# Autodesk Inventor assembly: HighFlowCO2Laser
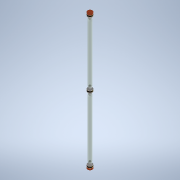
[picture p0: Inventor's stored thumbnail of the model, 180x180]
Saved by Autodesk Inventor 2020 (Build 240168000, 168)
## iProperties
Created: 2019-09-29
Part Number: HighFlowCO2Laser
Document SubType Name: Assembly
Designer: vmiguel
Author: vmiguel
## Documents named in this file (10)
- C:\Users\vmiguel\Documents\GitHub\HighFlowCO2Laser\HighFlowCO2Laser.iam
- C:\Users\vmiguel\Documents\GitHub\HighFlowCO2Laser\ZnSeWindow.ipt
- C:\Users\vmiguel\Documents\GitHub\HighFlowCO2Laser\GoldPlatedCopperMirror.ipt
- C:\Users\vmiguel\Documents\GitHub\HighFlowCO2Laser\TungstenFlange.ipt
- C:\Users\vmiguel\Documents\GitHub\HighFlowCO2Laser\CopperElectrode.ipt
- C:\Users\vmiguel\Documents\GitHub\HighFlowCO2Laser\MirrorHeatsink.ipt
- C:\Users\vmiguel\Documents\GitHub\HighFlowCO2Laser\InternalGlassTube.ipt
- C:\Users\vmiguel\Documents\GitHub\HighFlowCO2Laser\PTFESeal.ipt
- C:\Users\vmiguel\Documents\GitHub\HighFlowCO2Laser\Anode.ipt
- C:\Users\vmiguel\Documents\GitHub\HighFlowCO2Laser\OuterGlassTube.ipt
## Components (21 placed, 9 different names)
1. ZnSeWindow:1 — Mate:1, Mate:8, Mate:16
2. GoldPlatedCopperMirror:1 — Mate:1, Mate:48
3. TungstenFlange:1 — Mate:5, Mate:6, Mate:8, Mate:9, Mate:13, Mate:14, Mate:19, Mate:20, Mate:23, Mate:27
4. TungstenFlange:2 — Mate:2, Mate:3, Mate:4, Mate:5, Mate:6, Mate:9, Mate:12, Mate:33, Mate:34, Mate:35
5. TungstenFlange:3 — Mate:2, Mate:3, Mate:4, Mate:10, Mate:11, Mate:28, Mate:30, Mate:31, Mate:32
6. TungstenFlange:4 — Mate:10, Mate:11, Mate:12, Mate:29, Mate:38, Mate:39, Mate:40, Mate:42, Mate:43
7. CopperElectrode:1 — Mate:13, Mate:14, Mate:15, Mate:17, Mate:18, Mate:24, Mate:26
8. MirrorHeatsink:1 — Mate:15, Mate:16, Mate:17, Mate:18, Mate:21, Mate:22, Mate:25
9. InternalGlassTube:1 — Mate:19, Mate:20, Mate:36, Mate:50, Flush:3
10. PTFESeal:1 — Mate:21, Mate:22, Mate:25
11. PTFESeal:2 — Mate:23, Mate:24, Mate:26, Mate:27
12. InternalGlassTube:2 — Mate:28, Mate:29, Mate:51, Flush:4
13. PTFESeal:3 — Mate:30, Mate:31, Mate:32, Mate:37
14. PTFESeal:4 — Mate:33, Mate:34, Mate:35
15. Anode:1 — Mate:36, Mate:37
16. PTFESeal:5 — Mate:38, Mate:39, Mate:40, Mate:41
17. CopperElectrode:2 — Mate:41, Mate:42, Mate:43, Mate:44, Mate:45, Mate:46, Mate:49
18. PTFESeal:6 — Mate:44, Mate:45, Mate:46, Mate:47
19. MirrorHeatsink:2 — Mate:47, Mate:48, Mate:49
20. OuterGlassTube:1 — Mate:50, Flush:3
21. OuterGlassTube:2 — Mate:51, Flush:4
## Relationships (52: Mate 50, Flush 2)
- Mate:1: ZnSeWindow:1 ↔ GoldPlatedCopperMirror:1
- Mate:2 (14 mm): TungstenFlange:2 ↔ TungstenFlange:3
- Mate:3: TungstenFlange:2 ↔ TungstenFlange:3
- Mate:4: TungstenFlange:2 ↔ TungstenFlange:3
- Mate:5: TungstenFlange:1 ↔ TungstenFlange:2
- Mate:6: TungstenFlange:1 ↔ TungstenFlange:2
- Mate:8: ZnSeWindow:1 ↔ TungstenFlange:1
- Mate:9 (500 mm): TungstenFlange:1 ↔ TungstenFlange:2
- Mate:10 (500 mm): TungstenFlange:3 ↔ TungstenFlange:4
- Mate:11: TungstenFlange:3 ↔ TungstenFlange:4
- Mate:12: TungstenFlange:2 ↔ TungstenFlange:4
- Mate:13: TungstenFlange:1 ↔ CopperElectrode:1
- Mate:14 (2 mm): TungstenFlange:1 ↔ CopperElectrode:1
- Mate:15: CopperElectrode:1 ↔ MirrorHeatsink:1
- Mate:16: ZnSeWindow:1 ↔ MirrorHeatsink:1
- Mate:17 (2 mm): CopperElectrode:1 ↔ MirrorHeatsink:1
- Mate:18: CopperElectrode:1 ↔ MirrorHeatsink:1
- Mate:19: TungstenFlange:1 ↔ InternalGlassTube:1
- Mate:20 (10 mm): TungstenFlange:1 ↔ InternalGlassTube:1
- Mate:21: MirrorHeatsink:1 ↔ PTFESeal:1
- Mate:22: MirrorHeatsink:1 ↔ PTFESeal:1
- Mate:23: TungstenFlange:1 ↔ PTFESeal:2
- Mate:24: CopperElectrode:1 ↔ PTFESeal:2
- Mate:25: MirrorHeatsink:1 ↔ PTFESeal:1
- Mate:26: CopperElectrode:1 ↔ PTFESeal:2
- Mate:27: TungstenFlange:1 ↔ PTFESeal:2
- Mate:28: TungstenFlange:3 ↔ InternalGlassTube:2
- Mate:29 (10 mm): TungstenFlange:4 ↔ InternalGlassTube:2
- Mate:30: TungstenFlange:3 ↔ PTFESeal:3
- Mate:31: TungstenFlange:3 ↔ PTFESeal:3
- Mate:32: TungstenFlange:3 ↔ PTFESeal:3
- Mate:33: TungstenFlange:2 ↔ PTFESeal:4
- Mate:34: TungstenFlange:2 ↔ PTFESeal:4
- Mate:35: TungstenFlange:2 ↔ PTFESeal:4
- Mate:36: InternalGlassTube:1 ↔ Anode:1
- Mate:37: PTFESeal:3 ↔ Anode:1
- Mate:38: TungstenFlange:4 ↔ PTFESeal:5
- Mate:39: TungstenFlange:4 ↔ PTFESeal:5
- Mate:40: TungstenFlange:4 ↔ PTFESeal:5
- Mate:41: PTFESeal:5 ↔ CopperElectrode:2
- Mate:42: TungstenFlange:4 ↔ CopperElectrode:2
- Mate:43: TungstenFlange:4 ↔ CopperElectrode:2
- Mate:44: CopperElectrode:2 ↔ PTFESeal:6
- Mate:45: CopperElectrode:2 ↔ PTFESeal:6
- Mate:46: CopperElectrode:2 ↔ PTFESeal:6
- Mate:47: PTFESeal:6 ↔ MirrorHeatsink:2
- Mate:48: GoldPlatedCopperMirror:1 ↔ MirrorHeatsink:2
- Mate:49: CopperElectrode:2 ↔ MirrorHeatsink:2
- Mate:50: InternalGlassTube:1 ↔ OuterGlassTube:1
- Mate:51: InternalGlassTube:2 ↔ OuterGlassTube:2
- Flush:3 (-2 mm): InternalGlassTube:1 ↔ OuterGlassTube:1
- Flush:4 (2 mm): InternalGlassTube:2 ↔ OuterGlassTube:2
